# Autodesk Inventor assembly: v.3
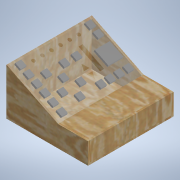
[picture p0: Inventor's stored thumbnail of the model, 180x180]
Saved by Autodesk Inventor 2021.1 (Build 251245000, 245)
## iProperties
Created: 2020-08-02
Part Number: v.3
Document SubType Name: Assembly
Designer: adick
Author: adick
## Documents named in this file (9)
- C:\Users\adick\Documents\Kerbal Kontroller\Design\Final\Inventor\Final.iam
- C:\Users\adick\Documents\Kerbal Kontroller\Design\Final\Inventor\Parts\Sides.ipt
- C:\Users\adick\Documents\Kerbal Kontroller\Design\Final\Inventor\Parts\Bottom.ipt
- C:\Users\adick\Documents\Kerbal Kontroller\Design\Final\Inventor\Parts\Front.ipt
- C:\Users\adick\Documents\Kerbal Kontroller\Design\Final\Inventor\Parts\Back.ipt
- C:\Users\adick\Documents\Kerbal Kontroller\Design\Final\Inventor\Parts\Plexi.ipt
- C:\Users\adick\Documents\Kerbal Kontroller\Design\Final\Inventor\Parts\Arm Rest.ipt
- C:\Users\adick\Documents\Kerbal Kontroller\Design\Final\Inventor\Parts\Stage Keycap.ipt
- C:\Users\adick\Documents\Kerbal Kontroller\Design\Final\Inventor\Parts\Keycaps.ipt
## Components (27 placed, 8 different names)
1. Sides:1 — Mate:8, Mate:9, Mate:11, Mate:64
2. Bottom:1 — Mate:2, Mate:10
3. Front:1 — Mate:1, Mate:9, Mate:10
4. Back:1 — Mate:11, Mate:63
5. Sides:2 — Mate:1, Mate:2, Mate:62
6. Plexi:1 — Mate:6, Mate:7, Mate:12, Mate:13, Mate:14, Mate:15, Mate:16, Mate:17, Mate:18, Mate:19, Mate:20, Mate:21, Mate:22, Mate:23, Mate:24, Mate:25, Mate:26, Mate:27, Mate:28, Mate:29, Mate:30, Mate:31, Mate:32, Mate:33, Mate:34, Mate:35, Mate:36, Mate:37, Mate:38, Mate:39, Mate:40, Mate:41, Mate:42, Mate:43, Mate:44, Mate:45, Mate:46, Mate:47, Mate:48, Mate:49, Mate:50, Mate:51, Mate:52, Mate:53, Mate:54, Mate:55, Mate:56, Mate:57, Mate:58, Mate:59, Mate:60, Mate:61, Mate:62, Mate:63, Mate:64
7. Arm Rest:1 — Mate:8
8. Stage Keycap:1 — Mate:6, Mate:7, Mate:12
9. Keycaps:3 — Mate:13, Mate:14, Mate:24
10. Keycaps:7 — Mate:15, Mate:16, Mate:23
11. Keycaps:8 — Mate:17, Mate:18, Mate:22
12. Keycaps:9 — Mate:56, Mate:57
13. Keycaps:10 — Mate:19, Mate:20, Mate:21
14. Keycaps:11 — Mate:52, Mate:53
15. Keycaps:12 — Mate:58, Mate:59
16. Keycaps:13 — Mate:50, Mate:51
17. Keycaps:14 — Mate:48, Mate:49
18. Keycaps:15 — Mate:34, Mate:35, Mate:39
19. Keycaps:16 — Mate:43, Mate:44, Mate:45
20. Keycaps:18 — Mate:54, Mate:55
21. Keycaps:19 — Mate:60, Mate:61
22. Keycaps:20 — Mate:28, Mate:29, Mate:30
23. Keycaps:21 — Mate:31, Mate:32, Mate:33
24. Keycaps:22 — Mate:36, Mate:37, Mate:38
25. Keycaps:23 — Mate:40, Mate:41, Mate:42
26. Keycaps:24 — Mate:46, Mate:47
27. Keycaps:25 — Mate:25, Mate:26, Mate:27
## Relationships (61: Mate 61)
- Mate:1: Front:1 ↔ Sides:2
- Mate:2: Bottom:1 ↔ Sides:2
- Mate:6: Plexi:1 ↔ Stage Keycap:1
- Mate:7: Plexi:1 ↔ Stage Keycap:1
- Mate:8: Sides:1 ↔ Arm Rest:1
- Mate:9: Sides:1 ↔ Front:1
- Mate:10: Bottom:1 ↔ Front:1
- Mate:11: Sides:1 ↔ Back:1
- Mate:12: Plexi:1 ↔ Stage Keycap:1
- Mate:13: Plexi:1 ↔ Keycaps:3
- Mate:14: Plexi:1 ↔ Keycaps:3
- Mate:15: Plexi:1 ↔ Keycaps:7
- Mate:16: Plexi:1 ↔ Keycaps:7
- Mate:17: Plexi:1 ↔ Keycaps:8
- Mate:18: Plexi:1 ↔ Keycaps:8
- Mate:19: Plexi:1 ↔ Keycaps:10
- Mate:20: Plexi:1 ↔ Keycaps:10
- Mate:21: Plexi:1 ↔ Keycaps:10
- Mate:22: Plexi:1 ↔ Keycaps:8
- Mate:23: Plexi:1 ↔ Keycaps:7
- Mate:24: Plexi:1 ↔ Keycaps:3
- Mate:25: Plexi:1 ↔ Keycaps:25
- Mate:26: Plexi:1 ↔ Keycaps:25
- Mate:27: Plexi:1 ↔ Keycaps:25
- Mate:28: Plexi:1 ↔ Keycaps:20
- Mate:29: Plexi:1 ↔ Keycaps:20
- Mate:30: Plexi:1 ↔ Keycaps:20
- Mate:31: Plexi:1 ↔ Keycaps:21
- Mate:32: Plexi:1 ↔ Keycaps:21
- Mate:33: Plexi:1 ↔ Keycaps:21
- Mate:34: Plexi:1 ↔ Keycaps:15
- Mate:35: Plexi:1 ↔ Keycaps:15
- Mate:36: Plexi:1 ↔ Keycaps:22
- Mate:37: Plexi:1 ↔ Keycaps:22
- Mate:38: Plexi:1 ↔ Keycaps:22
- Mate:39: Plexi:1 ↔ Keycaps:15
- Mate:40: Plexi:1 ↔ Keycaps:23
- Mate:41: Plexi:1 ↔ Keycaps:23
- Mate:42: Plexi:1 ↔ Keycaps:23
- Mate:43: Plexi:1 ↔ Keycaps:16
- Mate:44: Plexi:1 ↔ Keycaps:16
- Mate:45: Plexi:1 ↔ Keycaps:16
- Mate:46: Plexi:1 ↔ Keycaps:24
- Mate:47: Plexi:1 ↔ Keycaps:24
- Mate:48: Plexi:1 ↔ Keycaps:14
- Mate:49: Plexi:1 ↔ Keycaps:14
- Mate:50: Plexi:1 ↔ Keycaps:13
- Mate:51: Plexi:1 ↔ Keycaps:13
- Mate:52: Plexi:1 ↔ Keycaps:11
- Mate:53: Plexi:1 ↔ Keycaps:11
- Mate:54: Plexi:1 ↔ Keycaps:18
- Mate:55: Plexi:1 ↔ Keycaps:18
- Mate:56: Plexi:1 ↔ Keycaps:9
- Mate:57: Plexi:1 ↔ Keycaps:9
- Mate:58: Plexi:1 ↔ Keycaps:12
- Mate:59: Plexi:1 ↔ Keycaps:12
- Mate:60: Plexi:1 ↔ Keycaps:19
- Mate:61: Plexi:1 ↔ Keycaps:19
- Mate:62: Sides:2 ↔ Plexi:1
- Mate:63: Back:1 ↔ Plexi:1
- Mate:64: Sides:1 ↔ Plexi:1
